# Autodesk Inventor assembly: MMplates
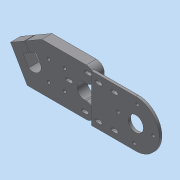
[picture p0: Inventor's stored thumbnail of the model, 180x180]
Saved by Autodesk Inventor 2017 (Build 210142000, 142)
## iProperties
Created: 2016-12-24
Part Number: MMplates
Document SubType Name: Assembly
Designer: Joshua Yuan
Author: Joshua Yuan
## Documents named in this file (3)
- C:\Other Project Stuff\Longboard\MMplates.iam
- C:\Other Project Stuff\Longboard\MMplate1.ipt
- C:\Other Project Stuff\Longboard\MMplate2.ipt
## Components (2 placed, 2 different names)
1. MMplate1:1 — Mate:1, Flush:1
2. MMplate2:1 — Mate:1, Flush:1
## Relationships (2: Mate 1, Flush 1)
- Mate:1: MMplate1:1 ↔ MMplate2:1
- Flush:1: MMplate1:1 ↔ MMplate2:1
